# Autodesk Inventor assembly: ASY GBK 1110 long wall shield 1
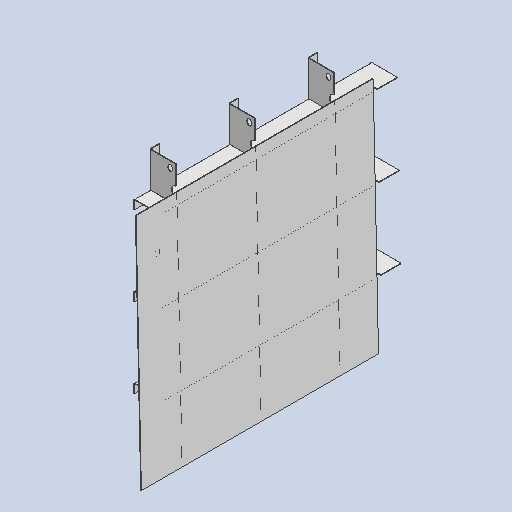
[picture p0: Inventor's stored thumbnail of the model, 512x512]
Saved by Autodesk Inventor 2026.3 (Build 303398000, 398)
## iProperties
Created: 2026-05-07
Part Number: ASY GBK 1110 long wall shield 1
Document SubType Name: Assembly
Designer: admin
Mass: 136093 g
Surface Area: 87957.2 cm^2
Volume: 17336.7 cm^3
Stock Number: 1110
Author: admin
Comments: поменял
## Documents named in this file (6)
- C:\Users\admin\Documents\Inventor\GBK-Gubkinskiy\ASY GBK 1110 long wall shield 1.iam
- C:\Users\admin\Documents\Inventor\GBK-Gubkinskiy\GBK 1115 shield 1.ipt
- C:\Users\admin\Documents\Inventor\GBK-Gubkinskiy\GBK 0101 main rib.ipt
- C:\Users\admin\Documents\Inventor\GBK-Gubkinskiy\GBK 0102 stringer 1.ipt
- C:\Users\admin\Documents\Inventor\GBK-Gubkinskiy\GBK 0103 stringer 2.ipt
- C:\Users\admin\Documents\Inventor\GBK-Gubkinskiy\GBK 0104 stringer 3.ipt
## Components (7 placed, 5 different names)
1. GBK 1115 shield 1:1 — Flush:5, Flush:6
2. GBK 0101 main rib:1 — Rigid:1, Rigid:2, Rigid:3, Mate:3, Mate:5
3. GBK 0102 stringer 1:1 — Rigid:1, Rigid:4, Rigid:5
4. GBK 0103 stringer 2:1 — Rigid:2, Flush:6
5. GBK 0104 stringer 3:1 — Rigid:3
6. GBK 0101 main rib:2 — Rigid:4
7. GBK 0101 main rib:3 — Rigid:5
## Relationships (11: WeldJoint 5, Mate 4, Flush 2)
- [Mate]: GBK 1115 shield 1:1 ↔ GBK 0101 main rib:1
- [Mate]: GBK 1115 shield 1:1 ↔ GBK 0101 main rib:1
- Rigid:1 [WeldJoint] (4 mm): GBK 0101 main rib:1 ↔ GBK 0102 stringer 1:1
- Rigid:2 [WeldJoint] (4 mm): GBK 0101 main rib:1 ↔ GBK 0103 stringer 2:1
- Rigid:3 [WeldJoint] (4 mm): GBK 0101 main rib:1 ↔ GBK 0104 stringer 3:1
- Mate:3: GBK 0101 main rib:1
- Flush:5: GBK 1115 shield 1:1
- Mate:5: GBK 0101 main rib:1
- Rigid:4 [WeldJoint] (4 mm): GBK 0102 stringer 1:1 ↔ GBK 0101 main rib:2
- Rigid:5 [WeldJoint] (4 mm): GBK 0102 stringer 1:1 ↔ GBK 0101 main rib:3
- Flush:6 (155 mm): GBK 1115 shield 1:1 ↔ GBK 0103 stringer 2:1
